# Autodesk Inventor assembly: A1-19027-500-00 Spool SP-235-002-D-002-1A
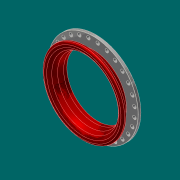
[picture p0: Inventor's stored thumbnail of the model, 180x180]
Saved by Autodesk Inventor 2017.3 (Build 213257000, 257)
## iProperties
Created: 2019-11-15
Part Number: A1-19027-500-00 Spool SP-235-002-D-002-1A
Document SubType Name: Assembly
Designer: GVD
Mass: 329433 g
Surface Area: 26173.7 cm^2
Volume: 44023 cm^3
Density: 7.48319 g/cm^3
Author: GVD
## Documents named in this file (3)
- N:\A1 - Projects\A1-19\A1-19027--Syncrude Aurora HT2 spools - SP-237\A1-19027-500-00 Spool SP-235-002-D-002-1A.iam
- N:\A1 - Projects\A1-19\A1-19027--Syncrude Aurora HT2 spools - SP-237\A1-19027-500-01 32in CL150 RF flange.ipt
- N:\A1 - Projects\A1-19\A1-19027--Syncrude Aurora HT2 spools - SP-237\A1-19028-500-02 HCWI nozzle horn.ipt
## Components (2 placed, 2 different names)
1. A1-19027-500-01 32in CL150 RF flange:1 — Mate:1, Mate:2, Angle:1, Insert:1, Angle:3
2. A1-19028-500-02 HCWI nozzle horn:1 — Insert:1, Angle:3
## Relationships (5: Mate 2, Angle 2, Insert 1)
- Mate:1: A1-19027-500-01 32in CL150 RF flange:1
- Mate:2: A1-19027-500-01 32in CL150 RF flange:1
- Angle:1 (0 deg): A1-19027-500-01 32in CL150 RF flange:1
- Insert:1: A1-19027-500-01 32in CL150 RF flange:1 ↔ A1-19028-500-02 HCWI nozzle horn:1
- Angle:3 (0 deg): A1-19027-500-01 32in CL150 RF flange:1 ↔ A1-19028-500-02 HCWI nozzle horn:1
